# Autodesk Inventor assembly: MK3_Assembly
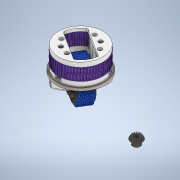
[picture p0: Inventor's stored thumbnail of the model, 180x180]
Saved by Autodesk Inventor 2020 (Build 240168000, 168)
## iProperties
Created: 2019-07-19
Part Number: MK3_Assembly
Document SubType Name: Assembly
Designer: Connor
Author: Connor
## Documents named in this file (12)
- C:\Users\Connor\Documents\GrabCAD\2019 Robot\Swerve\TorqyoDrift_MK3\MK3_Assembly.iam
- C:\Users\Connor\Documents\GrabCAD\2019 Robot\Swerve\TorqyoDrift_MK3\3inWheelHalf.ipt
- C:\Users\Connor\Documents\GrabCAD\2019 Robot\Swerve\TorqyoDrift_MK3\HubPlate.ipt
- C:\Users\Connor\Documents\GrabCAD\2019 Robot\Swerve\TorqyoDrift_MK3\BlueTread.ipt
- C:\Users\Connor\Documents\GrabCAD\2019 Robot\Swerve\TorqyoDrift_MK3\RingGear.iam
- C:\Users\Connor\Documents\GrabCAD\2019 Robot\Swerve\TorqyoDrift_MK3\PlanetCarriage.ipt
- C:\Users\Connor\Documents\GrabCAD\2019 Robot\Swerve\TorqyoDrift_MK3\Imported Components\Bearings\SA035XPO.ipt
- C:\Users\Connor\Documents\GrabCAD\2019 Robot\Swerve\TorqyoDrift_MK3\WheelBracketHead.ipt
- C:\Users\Connor\Documents\GrabCAD\2019 Robot\Swerve\TorqyoDrift_MK3\WheelBracketNut.ipt
- C:\Users\Connor\Documents\GrabCAD\2019 Robot\Swerve\TorqyoDrift_MK3\Bevel15t.ipt
- C:\Users\Connor\Documents\GrabCAD\2019 Robot\Swerve\TorqyoDrift_MK3\Bevel30t.ipt
- C:\Users\Connor\Documents\GrabCAD\2019 Robot\Swerve\TorqyoDrift_MK3\CarriageCap.ipt
## Components (14 placed, 11 different names)
1. 3inWheelHalf:1 — Insert:1, Mate:1, Insert:2, Mate:2, Insert:3, Mate:9, Mate:12, Mate:15
2. 3inWheelHalf:2 — Insert:2, Mate:2, Angle:1
3. HubPlate:1 — Insert:1, Mate:1
4. BlueTread:1 — Insert:3
5. RingGear:1 [sub-assembly] — Mate:3, Mate:4
6. RingGear:2 [sub-assembly] — Mate:3, Mate:4, Insert:7
7. PlanetCarriage:1 — Mate:8, Insert:4, Angle:1, Angle:2, Angle:3, Insert:7, Mate:15, Mate:16, Mate:17
8. SA035XPO:1 — Insert:4, Insert:5, Insert:6
9. WheelBracketHead:1 — Angle:2, Insert:5, Mate:9, Mate:10
10. WheelBracketNut:1 — Insert:6, Angle:3
11. Bevel15t:1
12. Bevel15t:2 — Mate:10, Mate:13, Mate:14
13. Bevel30t:1 — Mate:12, Mate:13, Mate:14
14. CarriageCap:1 — Mate:16, Mate:17
## Relationships (23: Mate 13, Insert 7, Angle 3)
- Insert:1: 3inWheelHalf:1 ↔ HubPlate:1
- Mate:1: 3inWheelHalf:1 ↔ HubPlate:1
- Insert:2: 3inWheelHalf:1 ↔ 3inWheelHalf:2
- Mate:2: 3inWheelHalf:1 ↔ 3inWheelHalf:2
- Insert:3: 3inWheelHalf:1 ↔ BlueTread:1
- Mate:3: RingGear:1 ↔ RingGear:2
- Mate:4: RingGear:1 ↔ RingGear:2
- Mate:8: PlanetCarriage:1
- Insert:4: PlanetCarriage:1 ↔ SA035XPO:1
- Angle:1 (0 deg): 3inWheelHalf:2 ↔ PlanetCarriage:1
- Angle:2 (0 deg): PlanetCarriage:1 ↔ WheelBracketHead:1
- Insert:5: SA035XPO:1 ↔ WheelBracketHead:1
- Insert:6: SA035XPO:1 ↔ WheelBracketNut:1
- Angle:3 (0 deg): PlanetCarriage:1 ↔ WheelBracketNut:1
- Mate:9: 3inWheelHalf:1 ↔ WheelBracketHead:1
- Insert:7: RingGear:2 ↔ PlanetCarriage:1
- Mate:10: WheelBracketHead:1 ↔ Bevel15t:2
- Mate:12: 3inWheelHalf:1 ↔ Bevel30t:1
- Mate:13 (-32 mm): Bevel15t:2 ↔ Bevel30t:1
- Mate:14 (-25 mm): Bevel15t:2 ↔ Bevel30t:1
- Mate:15 (3.175 mm): 3inWheelHalf:1 ↔ PlanetCarriage:1
- Mate:16: PlanetCarriage:1 ↔ CarriageCap:1
- Mate:17: PlanetCarriage:1 ↔ CarriageCap:1
